# Autodesk Inventor assembly: Shooter-Storage-IntakeAssembly.ver4-1111-2021
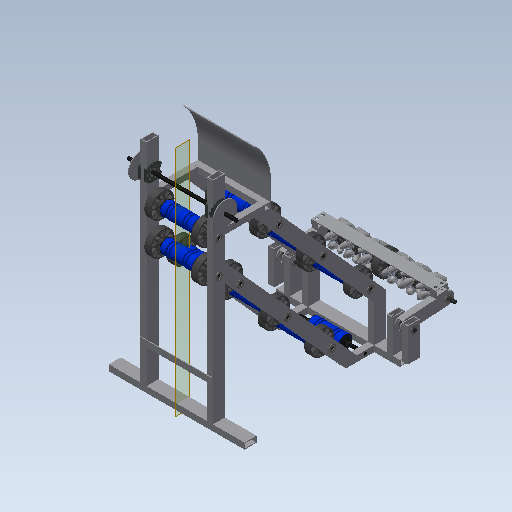
[picture p0: Inventor's stored thumbnail of the model, 512x512]
Saved by Autodesk Inventor 2021 (Build 250183000, 183)
## iProperties
Created: 2020-01-25
Part Number: Shooter-Storage-IntakeAssembly.ver4-1111-2021
Document SubType Name: Assembly
Designer: JMHal
Author: JMHal
## Documents named in this file (7)
- E:\PHRC CADD 2021\PHRC CADD\2020 Infinite Recharge\2021 Infinite Recharge\Chassis\Shooter-Storage-IntakeAssembly.ver4-1111-2021.iam
- E:\PHRC CADD 2021\PHRC CADD\2020 Infinite Recharge\Final Robot Assembly\IntakeAssembly-ver1-1111-2020.iam
- E:\PHRC CADD 2021\PHRC CADD\2020 Infinite Recharge\Shooting\Assemblies\ShooterPrototype-ver2-1111-2019.iam
- E:\PHRC CADD 2021\PHRC CADD\2020 Infinite Recharge\Storage\Assemblies\StorageAssembly.ver4-1111-2020.iam
- E:\PHRC CADD 2021\PHRC CADD\Resources\VEXpro Resources\Bearings\0.5inHexFlangedBearing(1.125inx0.313in)-1111-2016.ipt
- E:\PHRC CADD 2021\PHRC CADD\2020 Infinite Recharge\2021 Infinite Recharge\Chassis\Roller-ver4-1111-2021.iam
- E:\PHRC CADD 2021\PHRC CADD\2020 Infinite Recharge\2021 Infinite Recharge\Chassis\BottomRoller-ver1-1111-2021.iam
## Components (44 placed, 6 different names)
1. ShooterPrototype-ver2-1111-2019:1 [sub-assembly] — Mate:1, Flush:10, Mate:2, Mate:3, Rotational:27, Rotational:28, Rotational:29, Rotational:30, Rotational:31, Rotational:32, Rotational:33, Rotational:34, Flush:21
2. StorageAssembly.ver4-1111-2020:1 [sub-assembly] — Mate:1, Flush:10, Mate:2, Mate:3, Mate:4, Flush:11, Flush:12, Cylindrical:1, Mate:5, Cylindrical:2, Mate:6, Cylindrical:3, Mate:7, Rotational:1, Rotational:3, Rotational:4, Rotational:6, Rotational:7, Rotational:8, Rotational:10, Rotational:11, Rotational:12, Rotational:13, Rotational:14, Rotational:15, Rotational:16, Rotational:17, Rotational:19, Rotational:20, Rotational:21, Flush:13, Flush:15, Flush:16, Flush:17, Flush:18, Rotational:22, Rotational:23, Rotational:24, Rotational:25, Rotational:26, Flush:19, Flush:20
3. IntakeAssembly-ver1-1111-2020:2 [sub-assembly] — Mate:4, Flush:11, Flush:12
4. 0.5inHexFlangedBearing(1.125inx0.313in)-1111-2016:1 — Cylindrical:1, Mate:5
5. 0.5inHexFlangedBearing(1.125inx0.313in)-1111-2016:2 — Cylindrical:2, Mate:6
6. 0.5inHexFlangedBearing(1.125inx0.313in)-1111-2016:3 — Cylindrical:3, Mate:7
7. 0.5inHexFlangedBearing(1.125inx0.313in)-1111-2016:4 — Rotational:1, Cylindrical:4
8. 0.5inHexFlangedBearing(1.125inx0.313in)-1111-2016:5 — Rotational:3
9. 0.5inHexFlangedBearing(1.125inx0.313in)-1111-2016:6 — Rotational:23, Cylindrical:10
10. 0.5inHexFlangedBearing(1.125inx0.313in)-1111-2016:7 — Rotational:4
11. 0.5inHexFlangedBearing(1.125inx0.313in)-1111-2016:9 — Rotational:6
12. 0.5inHexFlangedBearing(1.125inx0.313in)-1111-2016:10 — Rotational:7, Cylindrical:9
13. 0.5inHexFlangedBearing(1.125inx0.313in)-1111-2016:11 — Rotational:8, Cylindrical:6
14. 0.5inHexFlangedBearing(1.125inx0.313in)-1111-2016:13 — Rotational:10, Cylindrical:8
15. 0.5inHexFlangedBearing(1.125inx0.313in)-1111-2016:14 — Rotational:11
16. 0.5inHexFlangedBearing(1.125inx0.313in)-1111-2016:15 — Rotational:12, Cylindrical:7
17. 0.5inHexFlangedBearing(1.125inx0.313in)-1111-2016:16 — Rotational:13
18. 0.5inHexFlangedBearing(1.125inx0.313in)-1111-2016:17 — Rotational:14
19. 0.5inHexFlangedBearing(1.125inx0.313in)-1111-2016:18 — Rotational:15
20. 0.5inHexFlangedBearing(1.125inx0.313in)-1111-2016:19 — Rotational:16
21. 0.5inHexFlangedBearing(1.125inx0.313in)-1111-2016:20 — Rotational:17
22. 0.5inHexFlangedBearing(1.125inx0.313in)-1111-2016:22 — Rotational:19
23. 0.5inHexFlangedBearing(1.125inx0.313in)-1111-2016:23 — Rotational:20
24. 0.5inHexFlangedBearing(1.125inx0.313in)-1111-2016:24 — Rotational:21
25. Roller-ver4-1111-2021:1 [sub-assembly] — Cylindrical:4, Flush:13
26. Roller-ver4-1111-2021:3 [sub-assembly] — Cylindrical:6, Flush:15
27. Roller-ver4-1111-2021:4 [sub-assembly] — Cylindrical:7, Flush:16
28. Roller-ver4-1111-2021:5 [sub-assembly] — Cylindrical:8, Flush:17
29. Roller-ver4-1111-2021:6 [sub-assembly] — Cylindrical:9, Flush:18
30. BottomRoller-ver1-1111-2021:1 [sub-assembly] — Rotational:22
31. 0.5inHexFlangedBearing(1.125inx0.313in)-1111-2016:25 — Rotational:24
32. 0.5inHexFlangedBearing(1.125inx0.313in)-1111-2016:26 — Rotational:25
33. 0.5inHexFlangedBearing(1.125inx0.313in)-1111-2016:27 — Rotational:26
34. Roller-ver4-1111-2021:7 [sub-assembly] — Cylindrical:10, Flush:19
35. 0.5inHexFlangedBearing(1.125inx0.313in)-1111-2016:28 — Rotational:27, Cylindrical:11
36. 0.5inHexFlangedBearing(1.125inx0.313in)-1111-2016:29 — Rotational:28
37. 0.5inHexFlangedBearing(1.125inx0.313in)-1111-2016:30 — Rotational:29
38. 0.5inHexFlangedBearing(1.125inx0.313in)-1111-2016:31 — Rotational:30
39. 0.5inHexFlangedBearing(1.125inx0.313in)-1111-2016:32 — Rotational:31
40. 0.5inHexFlangedBearing(1.125inx0.313in)-1111-2016:33 — Rotational:32, Cylindrical:12
41. 0.5inHexFlangedBearing(1.125inx0.313in)-1111-2016:34 — Rotational:33
42. 0.5inHexFlangedBearing(1.125inx0.313in)-1111-2016:35 — Rotational:34
43. Roller-ver4-1111-2021:8 [sub-assembly] — Cylindrical:11, Flush:20
44. Roller-ver4-1111-2021:9 [sub-assembly] — Cylindrical:12, Flush:21
## Relationships (59: RevoluteJoint 30, Flush 11, CylindricalJoint 11, Mate 7)
- Mate:1: ShooterPrototype-ver2-1111-2019:1 ↔ StorageAssembly.ver4-1111-2020:1
- Flush:10: ShooterPrototype-ver2-1111-2019:1 ↔ StorageAssembly.ver4-1111-2020:1
- Mate:2 (100.8888 mm): ShooterPrototype-ver2-1111-2019:1 ↔ StorageAssembly.ver4-1111-2020:1
- Mate:3: ShooterPrototype-ver2-1111-2019:1 ↔ StorageAssembly.ver4-1111-2020:1
- Mate:4: StorageAssembly.ver4-1111-2020:1 ↔ IntakeAssembly-ver1-1111-2020:2
- Flush:11: StorageAssembly.ver4-1111-2020:1 ↔ IntakeAssembly-ver1-1111-2020:2
- Flush:12 (-33.7185 mm): StorageAssembly.ver4-1111-2020:1 ↔ IntakeAssembly-ver1-1111-2020:2
- Cylindrical:1: StorageAssembly.ver4-1111-2020:1 ↔ 0.5inHexFlangedBearing(1.125inx0.313in)-1111-2016:1
- Mate:5: StorageAssembly.ver4-1111-2020:1 ↔ 0.5inHexFlangedBearing(1.125inx0.313in)-1111-2016:1
- Cylindrical:2: StorageAssembly.ver4-1111-2020:1 ↔ 0.5inHexFlangedBearing(1.125inx0.313in)-1111-2016:2
- Mate:6: StorageAssembly.ver4-1111-2020:1 ↔ 0.5inHexFlangedBearing(1.125inx0.313in)-1111-2016:2
- Cylindrical:3: StorageAssembly.ver4-1111-2020:1 ↔ 0.5inHexFlangedBearing(1.125inx0.313in)-1111-2016:3
- Mate:7: StorageAssembly.ver4-1111-2020:1 ↔ 0.5inHexFlangedBearing(1.125inx0.313in)-1111-2016:3
- Rotational:1 [RevoluteJoint]: StorageAssembly.ver4-1111-2020:1 ↔ 0.5inHexFlangedBearing(1.125inx0.313in)-1111-2016:4
- Rotational:3 [RevoluteJoint]: StorageAssembly.ver4-1111-2020:1 ↔ 0.5inHexFlangedBearing(1.125inx0.313in)-1111-2016:5
- Rotational:4 [RevoluteJoint]: StorageAssembly.ver4-1111-2020:1 ↔ 0.5inHexFlangedBearing(1.125inx0.313in)-1111-2016:7
- Rotational:6 [RevoluteJoint]: StorageAssembly.ver4-1111-2020:1 ↔ 0.5inHexFlangedBearing(1.125inx0.313in)-1111-2016:9
- Rotational:7 [RevoluteJoint]: StorageAssembly.ver4-1111-2020:1 ↔ 0.5inHexFlangedBearing(1.125inx0.313in)-1111-2016:10
- Rotational:8 [RevoluteJoint]: StorageAssembly.ver4-1111-2020:1 ↔ 0.5inHexFlangedBearing(1.125inx0.313in)-1111-2016:11
- Rotational:10 [RevoluteJoint]: StorageAssembly.ver4-1111-2020:1 ↔ 0.5inHexFlangedBearing(1.125inx0.313in)-1111-2016:13
- Rotational:11 [RevoluteJoint]: StorageAssembly.ver4-1111-2020:1 ↔ 0.5inHexFlangedBearing(1.125inx0.313in)-1111-2016:14
- Rotational:12 [RevoluteJoint]: StorageAssembly.ver4-1111-2020:1 ↔ 0.5inHexFlangedBearing(1.125inx0.313in)-1111-2016:15
- Rotational:13 [RevoluteJoint]: StorageAssembly.ver4-1111-2020:1 ↔ 0.5inHexFlangedBearing(1.125inx0.313in)-1111-2016:16
- Rotational:14 [RevoluteJoint]: StorageAssembly.ver4-1111-2020:1 ↔ 0.5inHexFlangedBearing(1.125inx0.313in)-1111-2016:17
- Rotational:15 [RevoluteJoint]: StorageAssembly.ver4-1111-2020:1 ↔ 0.5inHexFlangedBearing(1.125inx0.313in)-1111-2016:18
- Rotational:16 [RevoluteJoint]: StorageAssembly.ver4-1111-2020:1 ↔ 0.5inHexFlangedBearing(1.125inx0.313in)-1111-2016:19
- Rotational:17 [RevoluteJoint]: StorageAssembly.ver4-1111-2020:1 ↔ 0.5inHexFlangedBearing(1.125inx0.313in)-1111-2016:20
- Rotational:19 [RevoluteJoint]: StorageAssembly.ver4-1111-2020:1 ↔ 0.5inHexFlangedBearing(1.125inx0.313in)-1111-2016:22
- Rotational:20 [RevoluteJoint]: StorageAssembly.ver4-1111-2020:1 ↔ 0.5inHexFlangedBearing(1.125inx0.313in)-1111-2016:23
- Rotational:21 [RevoluteJoint]: StorageAssembly.ver4-1111-2020:1 ↔ 0.5inHexFlangedBearing(1.125inx0.313in)-1111-2016:24
- Cylindrical:4: 0.5inHexFlangedBearing(1.125inx0.313in)-1111-2016:4 ↔ Roller-ver4-1111-2021:1
- Flush:13: StorageAssembly.ver4-1111-2020:1 ↔ Roller-ver4-1111-2021:1
- Cylindrical:6: 0.5inHexFlangedBearing(1.125inx0.313in)-1111-2016:11 ↔ Roller-ver4-1111-2021:3
- Flush:15: StorageAssembly.ver4-1111-2020:1 ↔ Roller-ver4-1111-2021:3
- Cylindrical:7: 0.5inHexFlangedBearing(1.125inx0.313in)-1111-2016:15 ↔ Roller-ver4-1111-2021:4
- Flush:16: StorageAssembly.ver4-1111-2020:1 ↔ Roller-ver4-1111-2021:4
- Cylindrical:8: 0.5inHexFlangedBearing(1.125inx0.313in)-1111-2016:13 ↔ Roller-ver4-1111-2021:5
- Flush:17: StorageAssembly.ver4-1111-2020:1 ↔ Roller-ver4-1111-2021:5
- Cylindrical:9: 0.5inHexFlangedBearing(1.125inx0.313in)-1111-2016:10 ↔ Roller-ver4-1111-2021:6
- Flush:18: StorageAssembly.ver4-1111-2020:1 ↔ Roller-ver4-1111-2021:6
- Rotational:22 [RevoluteJoint]: StorageAssembly.ver4-1111-2020:1 ↔ BottomRoller-ver1-1111-2021:1
- Rotational:23 [RevoluteJoint]: StorageAssembly.ver4-1111-2020:1 ↔ 0.5inHexFlangedBearing(1.125inx0.313in)-1111-2016:6
- Rotational:24 [RevoluteJoint]: StorageAssembly.ver4-1111-2020:1 ↔ 0.5inHexFlangedBearing(1.125inx0.313in)-1111-2016:25
- Rotational:25 [RevoluteJoint]: StorageAssembly.ver4-1111-2020:1 ↔ 0.5inHexFlangedBearing(1.125inx0.313in)-1111-2016:26
- Rotational:26 [RevoluteJoint]: StorageAssembly.ver4-1111-2020:1 ↔ 0.5inHexFlangedBearing(1.125inx0.313in)-1111-2016:27
- Cylindrical:10: 0.5inHexFlangedBearing(1.125inx0.313in)-1111-2016:6 ↔ Roller-ver4-1111-2021:7
- Flush:19: StorageAssembly.ver4-1111-2020:1 ↔ Roller-ver4-1111-2021:7
- Rotational:27 [RevoluteJoint]: ShooterPrototype-ver2-1111-2019:1 ↔ 0.5inHexFlangedBearing(1.125inx0.313in)-1111-2016:28
- Rotational:28 [RevoluteJoint]: ShooterPrototype-ver2-1111-2019:1 ↔ 0.5inHexFlangedBearing(1.125inx0.313in)-1111-2016:29
- Rotational:29 [RevoluteJoint]: ShooterPrototype-ver2-1111-2019:1 ↔ 0.5inHexFlangedBearing(1.125inx0.313in)-1111-2016:30
- Rotational:30 [RevoluteJoint]: ShooterPrototype-ver2-1111-2019:1 ↔ 0.5inHexFlangedBearing(1.125inx0.313in)-1111-2016:31
- Rotational:31 [RevoluteJoint]: ShooterPrototype-ver2-1111-2019:1 ↔ 0.5inHexFlangedBearing(1.125inx0.313in)-1111-2016:32
- Rotational:32 [RevoluteJoint]: ShooterPrototype-ver2-1111-2019:1 ↔ 0.5inHexFlangedBearing(1.125inx0.313in)-1111-2016:33
- Rotational:33 [RevoluteJoint]: ShooterPrototype-ver2-1111-2019:1 ↔ 0.5inHexFlangedBearing(1.125inx0.313in)-1111-2016:34
- Rotational:34 [RevoluteJoint]: ShooterPrototype-ver2-1111-2019:1 ↔ 0.5inHexFlangedBearing(1.125inx0.313in)-1111-2016:35
- Cylindrical:11: 0.5inHexFlangedBearing(1.125inx0.313in)-1111-2016:28 ↔ Roller-ver4-1111-2021:8
- Flush:20: StorageAssembly.ver4-1111-2020:1 ↔ Roller-ver4-1111-2021:8
- Cylindrical:12: 0.5inHexFlangedBearing(1.125inx0.313in)-1111-2016:33 ↔ Roller-ver4-1111-2021:9
- Flush:21: ShooterPrototype-ver2-1111-2019:1 ↔ Roller-ver4-1111-2021:9
